# Autodesk Inventor assembly: disposição_chapa
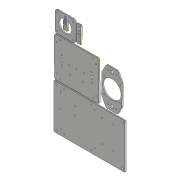
[picture p0: Inventor's stored thumbnail of the model, 180x180]
Saved by Autodesk Inventor 2020 (Build 240168000, 168)
## iProperties
Created: 2022-07-24
Part Number: disposição_chapa
Document SubType Name: Assembly
Designer: gabri
Author: gabri
## Documents named in this file (7)
- C:\Users\gabri\OneDrive\Área de Trabalho\Calorimetro 2022\Inventor\disposição_chapa.iam
- C:\Users\gabri\OneDrive\Área de Trabalho\Calorimetro 2022\Inventor\Base.ipt
- C:\Users\gabri\OneDrive\Área de Trabalho\Calorimetro 2022\Inventor\fechamentocima.ipt
- C:\Users\gabri\OneDrive\Área de Trabalho\Calorimetro 2022\Inventor\Suporte_inferior_menor.ipt
- C:\Users\gabri\OneDrive\Área de Trabalho\Calorimetro 2022\Inventor\Suporte_superior_menor.ipt
- C:\Users\gabri\OneDrive\Área de Trabalho\Calorimetro 2022\Inventor\suporte_termopar_al.ipt
- C:\Users\gabri\OneDrive\Área de Trabalho\Calorimetro 2022\Inventor\tampa_suporte_termopar.ipt
## Components (6 placed, 6 different names)
1. Base:1 — Alinhamento:1, Alinhamento:2
2. fechamentocima:1 — Alinhamento:1
3. Suporte_inferior_menor:1 — Alinhamento:2, Alinhamento:3, Alinhamento:4, Alinhamento:5
4. Suporte_superior_menor:1 — Alinhamento:3
5. suporte_termopar_al:1 — Alinhamento:4
6. tampa_suporte_termopar:1 — Alinhamento:5
## Relationships (5: Flush 5)
- Alinhamento:1 [Flush]: Base:1 ↔ fechamentocima:1
- Alinhamento:2 [Flush]: Base:1 ↔ Suporte_inferior_menor:1
- Alinhamento:3 [Flush]: Suporte_inferior_menor:1 ↔ Suporte_superior_menor:1
- Alinhamento:4 [Flush]: Suporte_inferior_menor:1 ↔ suporte_termopar_al:1
- Alinhamento:5 [Flush]: Suporte_inferior_menor:1 ↔ tampa_suporte_termopar:1
